# Autodesk Inventor assembly: Placed 90 deg corner cabinet door
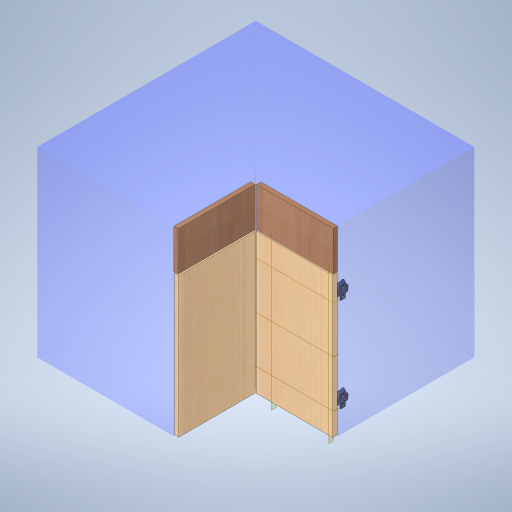
[picture p0: Inventor's stored thumbnail of the model, 512x512]
Saved by Autodesk Inventor 2024 (Build 280153000, 153)
## iProperties
RuleStatus: InUse
Created: 2017-01-31
Part Number: Placed 90 deg corner cabinet door
Document SubType Name: Assembly
Designer: SvetlanaB
Author: SvetlanaB
## Documents named in this file (8)
- C:\W4INV 2024 Design\iBOX LIBRARY\Kitchen\Doors\Corner cabinet door L type\Corner cabinet door L type.iam
- C:\W4INV 2024 Design\iBOX LIBRARY\Kitchen\Doors\Corner cabinet door L type\Drawer facade.ipt
- C:\W4INV 2024 Design\iBOX LIBRARY\Kitchen\Doors\Corner cabinet door L type\Right door.ipt
- C:\W4INV 2024 Design\iBOX LIBRARY\Kitchen\Doors\Corner cabinet door L type\Drawer facade_2.ipt
- C:\W4INV 2024 Design\iBOX LIBRARY\Kitchen\Doors\Corner cabinet door L type\Left door.ipt
- C:\W4INV 2024 Design\_LIBRARY\Hinges\170 DEGREE HINGE\170 Degree Hinge with Wood Screws And Cup Fixing Wood Screws.iam
- C:\W4INV 2024 Design\iBOX LIBRARY\Kitchen\Doors\Corner cabinet door L type\cab door con.ipt
- C:\W4INV 2023 Design\LIBRARY\Hinges\170 DEGREE HINGE.iam
## Components (7 placed, 6 different names)
1. Drawer facade:1
2. Right door:1 — Mate:3, Mate:4, Flush:9, Mate:5, Angle:1, Flush:10, Flush:11, Flush:12
3. Drawer facade_2:1
4. Left door:1
5. 170 Degree Hinge with Wood Screws And Cup Fixing Wood Screws:1 [sub-assembly] — Mate:3, Flush:6, Mate:10
6. 170 Degree Hinge with Wood Screws And Cup Fixing Wood Screws:2 [sub-assembly] — Mate:4, Flush:7, Mate:9
7. @cab door con:1
## Relationships (12: Flush 6, Mate 5, Angle 1)
- Mate:3: Right door:1 ↔ 170 Degree Hinge with Wood Screws And Cup Fixing Wood Screws:1
- Flush:6: 170 Degree Hinge with Wood Screws And Cup Fixing Wood Screws:1
- Mate:4: Right door:1 ↔ 170 Degree Hinge with Wood Screws And Cup Fixing Wood Screws:2
- Flush:7: 170 Degree Hinge with Wood Screws And Cup Fixing Wood Screws:2
- Flush:9 (-64 mm): Right door:1
- Mate:5: Right door:1
- Angle:1 (0 deg): Right door:1
- Flush:10 (-96 mm): Right door:1
- Flush:11 (-96 mm): Right door:1
- Mate:9: 170 Degree Hinge with Wood Screws And Cup Fixing Wood Screws:2
- Mate:10: 170 Degree Hinge with Wood Screws And Cup Fixing Wood Screws:1
- Flush:12 (-15 mm): Right door:1
## Named parameters: Side_allowance = 3 mm, Panel_thickness = 18 mm
